# Autodesk Inventor assembly: torso
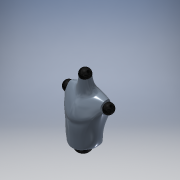
[picture p0: Inventor's stored thumbnail of the model, 180x180]
Saved by Autodesk Inventor 2018 (Build 220112000, 112)
## iProperties
Created: 2020-03-01
Part Number: torso
Document SubType Name: Assembly
Designer: Matt
Author: Matt
## Documents named in this file (2)
- C:\Users\Matt\robot\multibodySim\human\Corpo Humano - ADEBOTT Projetos\torso.iam
- C:\Users\Matt\robot\multibodySim\human\Corpo Humano - ADEBOTT Projetos\01.02.01.01 - Torso.ipt
## Components (1 placed, 1 different names)
1. 01.02.01.01 - Torso:1 — Tangent:1, Tangent:2, Tangent:3
## Relationships (10: Angle 3, Tangent 3, Mate 3, Flush 1)
- Angle:1 (0 deg)
- Tangent:1: 01.02.01.01 - Torso:1
- Angle:2 (0 deg)
- Tangent:2: 01.02.01.01 - Torso:1
- Angle:3 (0 deg)
- Tangent:3: 01.02.01.01 - Torso:1
- Mate:1 (-50 mm)
- Mate:2 (-50 mm)
- Mate:3 (-50 mm)
- Flush:1 (-50 mm)
